# Autodesk Inventor assembly: Frame 1647030135921
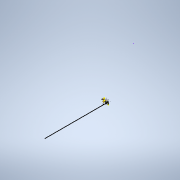
[picture p0: Inventor's stored thumbnail of the model, 180x180]
Saved by Autodesk Inventor 2022.2 (Build 262287010, 287A)
## iProperties
Created: 2022-03-11
Part Number: Frame 1647030135921
Document SubType Name: Assembly
Designer: foriw
Mass: 3267.05 g
Surface Area: 4067.66 cm^2
Volume: 419.019 cm^3
Density: 7.79691 g/cm^3
_FrameDoc: Frame Assembly
_Version: 25.0.0
Author: foriw
## Documents named in this file (36)
- C:\Users\Finn Oriwohl\Documents\htx\1g g\BeerCart-CAD-Inventor\Workspaces\Workspace\beercart assembly - mekatronik\Frame\Frame 1647030135921.iam
- C:\Users\Finn Oriwohl\Documents\htx\1g g\BeerCart-CAD-Inventor\Workspaces\Workspace\beercart assembly - mekatronik\Frame\Skeleton 1647030135922.ipt
- C:\Users\Finn Oriwohl\Documents\htx\1g g\BeerCart-CAD-Inventor\Workspaces\Workspace\beercart assembly - mekatronik\Frame\ISO 12633-2 20x20x2 1647030137505.ipt
- C:\Users\Finn Oriwohl\Documents\htx\1g g\BeerCart-CAD-Inventor\Workspaces\Workspace\beercart assembly - mekatronik\Frame\ISO 12633-2 20x20x2 1647030138110.ipt
- C:\Users\Finn Oriwohl\Documents\htx\1g g\BeerCart-CAD-Inventor\Workspaces\Workspace\beercart assembly - mekatronik\Frame\ISO 12633-2 20x20x2 1647030138225.ipt
- C:\Users\Finn Oriwohl\Documents\htx\1g g\BeerCart-CAD-Inventor\Workspaces\Workspace\beercart assembly - mekatronik\Frame\ISO 12633-2 20x20x2 1647030639616.ipt
- C:\Users\Finn Oriwohl\Documents\htx\1g g\BeerCart-CAD-Inventor\Workspaces\Workspace\beercart assembly - mekatronik\Frame\ISO 12633-2 20x20x2 1647030639707.ipt
- C:\Users\Finn Oriwohl\Documents\htx\1g g\BeerCart-CAD-Inventor\Workspaces\Workspace\beercart assembly - mekatronik\Frame\ISO 1035_2 10x 10 1647602096505.ipt
- C:\Users\Finn Oriwohl\Documents\htx\1g g\BeerCart-CAD-Inventor\Workspaces\Workspace\beercart assembly - mekatronik\Frame\ISO 1035_2 10x 10 1647602096566.ipt
- C:\Users\Finn Oriwohl\Documents\htx\1g g\BeerCart-CAD-Inventor\Workspaces\Workspace\beercart assembly - mekatronik\Frame\ISO 1035_2 10x 10 1647602096620.ipt
- C:\Users\Finn Oriwohl\Documents\htx\1g g\BeerCart-CAD-Inventor\Workspaces\Workspace\beercart assembly - mekatronik\Frame\ISO 12633-2 20x20x2 1647606177319.ipt
- C:\Users\Finn Oriwohl\Documents\htx\1g g\BeerCart-CAD-Inventor\Workspaces\Workspace\beercart assembly - mekatronik\Frame\ISO 12633-2 20x20x2 1647606177438.ipt
- C:\Users\Finn Oriwohl\Documents\htx\1g g\BeerCart-CAD-Inventor\Workspaces\Workspace\BackWheelMountingPlate.ipt
- C:\Users\Finn Oriwohl\Documents\htx\1g g\BeerCart-CAD-Inventor\Workspaces\Workspace\BackWheelMountingPlate_MIR_MIR.ipt
- C:\Users\Finn Oriwohl\Documents\htx\1g g\BeerCart-CAD-Inventor\Workspaces\Workspace\beercart assembly - mekatronik\Frame\ISO 1035_2 10x 10 1648211737860.ipt
- C:\Users\Finn Oriwohl\Documents\htx\1g g\BeerCart-CAD-Inventor\Workspaces\Workspace\bearing housing front.ipt
- C:\Users\Finn Oriwohl\Documents\htx\1g g\BeerCart-CAD-Inventor\Workspaces\Workspace\beercart assembly - mekatronik\Frame\ISO 12633-2 20x20x2 1648573909221.ipt
- C:\Users\Finn Oriwohl\Documents\htx\1g g\BeerCart-CAD-Inventor\Workspaces\Workspace\beercart assembly - mekatronik\Frame\ISO 12633-2 20x20x2 1648573975084.ipt
- C:\Users\Finn Oriwohl\Documents\htx\1g g\BeerCart-CAD-Inventor\Workspaces\Workspace\beercart assembly - mekatronik\Frame\ISO 12633-2 20x20x2 1648627088055.ipt
- C:\Users\Finn Oriwohl\Documents\htx\1g g\BeerCart-CAD-Inventor\Workspaces\Workspace\beercart assembly - mekatronik\Frame\ISO 12633-2 20x20x2 1648627088175.ipt
- C:\Users\Finn Oriwohl\Documents\htx\1g g\BeerCart-CAD-Inventor\Workspaces\Workspace\BackWheelMountingPlate_MIR4.ipt
- C:\Users\Finn Oriwohl\Documents\htx\1g g\BeerCart-CAD-Inventor\Workspaces\Workspace\beercart assembly - mekatronik\Frame\ISO 12633-2 20x20x2 1648631331581.ipt
- C:\Users\Finn Oriwohl\Documents\htx\1g g\BeerCart-CAD-Inventor\Workspaces\Workspace\beercart assembly - mekatronik\Frame\ISO 12633-2 20x20x2 1649085652950.ipt
- C:\Users\Finn Oriwohl\Documents\htx\1g g\BeerCart-CAD-Inventor\Workspaces\Workspace\beercart assembly - mekatronik\Frame\ISO 12633-2 20x20x2 1649085653040.ipt
- C:\Users\Finn Oriwohl\Documents\htx\1g g\BeerCart-CAD-Inventor\Workspaces\Workspace\backWheelNoMotor brake mount.ipt
- C:\Users\Finn Oriwohl\Documents\htx\1g g\BeerCart-CAD-Inventor\Workspaces\Workspace\beercart assembly - mekatronik\Frame\ISO 12633-2 20x20x2 1649154464355.ipt
- C:\Users\Finn Oriwohl\Documents\htx\1g g\BeerCart-CAD-Inventor\Workspaces\Workspace\BackWheelMotorMountSpacer.ipt
- C:\Users\Finn Oriwohl\Documents\htx\1g g\BeerCart-CAD-Inventor\Workspaces\Workspace\beercart assembly - mekatronik\Frame\FrontWheelFrameNew.iam
- C:\Users\Finn Oriwohl\Documents\htx\1g g\BeerCart-CAD-Inventor\Workspaces\Workspace\FrontWheelAssembly.iam
- C:\Users\Finn Oriwohl\Documents\htx\1g g\BeerCart-CAD-Inventor\Workspaces\Workspace\beercart assembly - mekatronik\Frame\ISO 12633-2 20x20x2 1649404567614.ipt
- C:\Users\Finn Oriwohl\Documents\htx\1g g\BeerCart-CAD-Inventor\Workspaces\Workspace\beercart assembly - mekatronik\Frame\ISO 12633-2 20x20x2 1649404567728.ipt
- C:\Users\Finn Oriwohl\Documents\htx\1g g\BeerCart-CAD-Inventor\Workspaces\Workspace\beercart assembly - mekatronik\Frame\ISO 12633-2 20x20x2 1649404567852.ipt
- C:\Users\Finn Oriwohl\Documents\htx\1g g\BeerCart-CAD-Inventor\Workspaces\Workspace\beercart assembly - mekatronik\Frame\ISO 12633-2 20x20x2 1649404567971.ipt
- C:\Users\Finn Oriwohl\Documents\htx\1g g\BeerCart-CAD-Inventor\Workspaces\Workspace\beercart assembly - mekatronik\Frame\ISO 12633-2 20x20x2 1649404568085.ipt
- C:\Users\Finn Oriwohl\Documents\htx\1g g\BeerCart-CAD-Inventor\Workspaces\Workspace\beercart assembly - mekatronik\Frame\ISO 12633-2 20x20x2 1649404568198.ipt
- C:\Users\Finn Oriwohl\Documents\htx\1g g\BeerCart-CAD-Inventor\Workspaces\Workspace\beercart assembly - mekatronik\Frame\ISO 12633-2 20x20x2 1649404611702.ipt
## Components (35 placed, 26 different names)
1. bearing housing front:1 — Insert:1
2. Reference Skeleton
3. ISO 12633-2 20x20x2 - 319.23:2
4. ISO 12633-2 20x20x2 - 290:1
5. ISO 12633-2 20x20x2 - 159.94:3
6. ISO 12633-2 20x20x2 - 182.18:1
7. ISO 12633-2 20x20x2 - 182.18:2
8. ISO 1035/2 10x 10 - 58.08:1
9. ISO 1035/2 10x 10 - 68.33:1
10. ISO 1035/2 10x 10 - 68.33:2
11. ISO 12633-2 20x20x2 - 152.97:1 — Mate:1, Mate:3
12. ISO 12633-2 20x20x2 - 152.97:2 — Mate:2, Mate:4, Mate:5
13. BackWheelMountingPlate:1 — Flush:6, Rotational:2, Rigid:1
14. BackWheelMountingPlate_MIR_MIR:1
15. ISO 1035/2 10x 10 - 58.08:1
16. ISO 12633-2 20x20x2 - 282.98:1
17. ISO 12633-2 20x20x2 - 44,58:1 — Flush:6, Rotational:2, Rigid:1
18. ISO 12633-2 20x20x2 - 33,46:1 — Rotational:5, Flush:9, Flush:11, Flush:12, Flush:13
19. ISO 12633-2 20x20x2 - 98,7:1
20. BackWheelMountingPlate_MIR4:1 — Rotational:5, Flush:9
21. ISO 12633-2 20x20x2 - 282.98:1
22. ISO 12633-2 20x20x2 - 98.7:1
23. ISO 12633-2 20x20x2 - 33,46:1 — Flush:10
24. backWheelNoMotor brake mount:1 — Flush:10
25. ISO 12633-2 20x20x2 - 44.58:1
26. BackWheelMotorMountSpacer:1 — Flush:11, Flush:12, Flush:13
27. FrontWheelFrameNew:1 [sub-assembly] — Insert:1
28. FrontWheelAssembly:1 [sub-assembly]
29. ISO 12633-2 20x20x2 - 245.2:1
30. ISO 12633-2 20x20x2 - 258.05:2
31. ISO 12633-2 20x20x2 - 258.05:3
32. ISO 12633-2 20x20x2 - 245.2:4
33. ISO 12633-2 20x20x2 - 90.41:1
34. ISO 12633-2 20x20x2 - 90.41:2
35. ISO 12633-2 20x20x2 - 65:3
## Relationships (19: Flush 7, Mate 6, Insert 3, RevoluteJoint 2, WeldJoint 1)
- Mate:1: ISO 12633-2 20x20x2 - 152.97:1
- Mate:2: ISO 12633-2 20x20x2 - 152.97:2
- Mate:3: ISO 12633-2 20x20x2 - 152.97:1
- Mate:4: ISO 12633-2 20x20x2 - 152.97:2
- Mate:5: ISO 12633-2 20x20x2 - 152.97:2
- [Mate]: bearing housing front:1 ↔ ISO 1035/2 10x 10 - 58.08:1
- [Flush]: bearing housing front:1 ↔ ISO 1035/2 10x 10 - 58.08:1
- Flush:6: BackWheelMountingPlate:1 ↔ ISO 12633-2 20x20x2 - 44,58:1
- Rotational:2 [RevoluteJoint]: BackWheelMountingPlate:1 ↔ ISO 12633-2 20x20x2 - 44,58:1
- Rotational:5 [RevoluteJoint]: ISO 12633-2 20x20x2 - 33,46:1 ↔ BackWheelMountingPlate_MIR4:1
- Flush:9: ISO 12633-2 20x20x2 - 33,46:1 ↔ BackWheelMountingPlate_MIR4:1
- Flush:10: ISO 12633-2 20x20x2 - 33,46:1 ↔ backWheelNoMotor brake mount:1
- Rigid:1 [WeldJoint]: BackWheelMountingPlate:1 ↔ ISO 12633-2 20x20x2 - 44,58:1
- Flush:11: ISO 12633-2 20x20x2 - 33,46:1 ↔ BackWheelMotorMountSpacer:1
- Flush:12: ISO 12633-2 20x20x2 - 33,46:1 ↔ BackWheelMotorMountSpacer:1
- Flush:13: ISO 12633-2 20x20x2 - 33,46:1 ↔ BackWheelMotorMountSpacer:1
- Insert:1 (2 mm): bearing housing front:1 ↔ FrontWheelFrameNew:1
- [Insert]: FrontWheelFrameNew:1 ↔ FrontWheelAssembly:1
- [Insert]: FrontWheelFrameNew:1 ↔ FrontWheelAssembly:1
## Named parameters: d22_d2 = 0 mm, d23_d3 = 0 mm, d59_d44 = 0 mm
